# Autodesk Inventor assembly: BaseMini
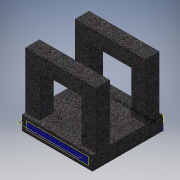
[picture p0: Inventor's stored thumbnail of the model, 180x180]
Saved by Autodesk Inventor 2016 (Build 200138000, 138)
## iProperties
Created: 2015-08-01
Part Number: BaseMini
Document SubType Name: Assembly
Designer: myhome
Author: myhome
## Documents named in this file (3)
- C:\Users\myhome\Documents\Inventor\Printer\EpoxyGraniteBase\BaseMini.iam
- C:\Users\myhome\Documents\Inventor\Printer\EpoxyGraniteBase\BaseMini.ipt
- C:\Users\myhome\Documents\Inventor\Printer\EpoxyGraniteBase\RailsMini.ipt
## Components (3 placed, 2 different names)
1. BaseMini:1 — Flush:1, Flush:2, Flush:3, Mate:1, Mate:2, Mate:3, Mate:4
2. RailsMini:1 — Mate:1, Mate:2
3. RailsMini:2 — Mate:3, Mate:4
## Relationships (7: Mate 4, Flush 3)
- Flush:1: BaseMini:1
- Flush:2: BaseMini:1
- Flush:3: BaseMini:1
- Mate:1: BaseMini:1 ↔ RailsMini:1
- Mate:2: BaseMini:1 ↔ RailsMini:1
- Mate:3: BaseMini:1 ↔ RailsMini:2
- Mate:4: BaseMini:1 ↔ RailsMini:2
